# Autodesk Inventor assembly: platform
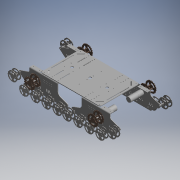
[picture p0: Inventor's stored thumbnail of the model, 180x180]
Saved by Autodesk Inventor 2019.4 (Build 234330000, 330)
## iProperties
Part Number: platform
Document SubType Name: Assembly
Designer: Jorge
Author: Jorge
## Documents named in this file (7)
- D:\TFG\dev\hardware\ROVER\platform.iam
- D:\TFG\dev\hardware\ROVER\platform_board.ipt
- D:\TFG\dev\hardware\ROVER\platform_track_support.ipt
- D:\TFG\dev\hardware\ROVER\platform_track_support_inv.ipt
- D:\TFG\dev\hardware\ROVER\platform_motor.ipt
- D:\TFG\dev\hardware\ROVER\platform_wheel.ipt
- D:\TFG\dev\hardware\ROVER\platform_sprocket.ipt
## Components (33 placed, 6 different names)
1. platform_board:1 — Mate:1, Mate:2, Mate:3, Mate:4, Mate:5, Mate:6, Mate:7, Mate:8, Mate:9, Mate:10, Mate:11, Mate:12, Mate:25, Mate:26, Mate:27
2. platform_track_support:1 — Mate:3, Mate:9, Mate:10, Mate:18, Mate:19, Mate:20, Mate:36, Mate:37, Mate:38, Mate:39, Mate:40, Mate:41, Mate:42, Mate:43, Mate:46, Mate:47
3. platform_track_support:2 — Mate:1, Mate:5, Mate:6, Mate:21, Mate:22, Mate:23, Mate:53, Mate:54, Mate:55, Mate:56, Mate:57, Mate:63, Mate:64, Mate:65, Mate:66, Mate:67
4. platform_track_support_inv:1 — Mate:4, Mate:7, Mate:8, Mate:13, Mate:14, Mate:15, Mate:48, Mate:49, Mate:50, Mate:51, Mate:52, Mate:58, Mate:59, Mate:60, Mate:61, Mate:62
5. platform_track_support_inv:2 — Mate:2, Mate:11, Mate:12, Mate:16, Mate:17, Mate:24, Mate:28, Mate:29, Mate:30, Mate:31, Mate:32, Mate:33, Mate:34, Mate:35, Mate:44, Mate:45
6. platform_motor:1 — Mate:13, Mate:14, Mate:15, Mate:71, Mate:72
7. platform_motor:2 — Mate:18, Mate:19, Mate:20, Mate:69, Mate:70
8. platform_motor:3 — Mate:16, Mate:17, Mate:24, Mate:74, Flush:1
9. platform_motor:4 — Mate:21, Mate:22, Mate:23, Mate:73
10. platform_wheel:1 — Mate:28, Mate:29
11. platform_wheel:2 — Mate:31, Mate:34
12. platform_wheel:3 — Mate:30, Mate:35
13. platform_wheel:4 — Mate:32, Mate:33
14. platform_wheel:5 — Mate:36, Mate:37
15. platform_wheel:6 — Mate:38, Mate:41
16. platform_wheel:7 — Mate:39, Mate:42
17. platform_wheel:8 — Mate:40, Mate:43
18. platform_wheel:9 — Mate:46, Mate:47
19. platform_wheel:10 — Mate:44, Mate:45
20. platform_wheel:11 — Mate:49, Mate:59
21. platform_wheel:12 — Mate:50, Mate:60
22. platform_wheel:13 — Mate:51, Mate:61
23. platform_wheel:14 — Mate:52, Mate:62
24. platform_wheel:15 — Mate:53, Mate:67
25. platform_wheel:16 — Mate:54, Mate:66
26. platform_wheel:17 — Mate:55, Mate:65
27. platform_wheel:18 — Mate:56, Mate:64
28. platform_wheel:19 — Mate:57, Mate:63
29. platform_wheel:20 — Mate:48, Mate:58
30. platform_sprocket:1 — Mate:74, Flush:1
31. platform_sprocket:2 — Mate:69, Mate:70
32. platform_sprocket:3 — Mate:71, Mate:72
33. platform_sprocket:4 — Mate:73
## Relationships (74: Mate 73, Flush 1)
- Mate:1: platform_board:1 ↔ platform_track_support:2
- Mate:2: platform_board:1 ↔ platform_track_support_inv:2
- Mate:3: platform_board:1 ↔ platform_track_support:1
- Mate:4: platform_board:1 ↔ platform_track_support_inv:1
- Mate:5: platform_board:1 ↔ platform_track_support:2
- Mate:6: platform_board:1 ↔ platform_track_support:2
- Mate:7: platform_board:1 ↔ platform_track_support_inv:1
- Mate:8: platform_board:1 ↔ platform_track_support_inv:1
- Mate:9: platform_board:1 ↔ platform_track_support:1
- Mate:10: platform_board:1 ↔ platform_track_support:1
- Mate:11: platform_board:1 ↔ platform_track_support_inv:2
- Mate:12: platform_board:1 ↔ platform_track_support_inv:2
- Mate:13: platform_track_support_inv:1 ↔ platform_motor:1
- Mate:14: platform_track_support_inv:1 ↔ platform_motor:1
- Mate:15: platform_track_support_inv:1 ↔ platform_motor:1
- Mate:16: platform_track_support_inv:2 ↔ platform_motor:3
- Mate:17: platform_track_support_inv:2 ↔ platform_motor:3
- Mate:18: platform_track_support:1 ↔ platform_motor:2
- Mate:19: platform_track_support:1 ↔ platform_motor:2
- Mate:20: platform_track_support:1 ↔ platform_motor:2
- Mate:21: platform_track_support:2 ↔ platform_motor:4
- Mate:22: platform_track_support:2 ↔ platform_motor:4
- Mate:23: platform_track_support:2 ↔ platform_motor:4
- Mate:24: platform_track_support_inv:2 ↔ platform_motor:3
- Mate:25: platform_board:1
- Mate:26: platform_board:1
- Mate:27: platform_board:1
- Mate:28: platform_track_support_inv:2 ↔ platform_wheel:1
- Mate:29: platform_track_support_inv:2 ↔ platform_wheel:1
- Mate:30: platform_track_support_inv:2 ↔ platform_wheel:3
- Mate:31: platform_track_support_inv:2 ↔ platform_wheel:2
- Mate:32: platform_track_support_inv:2 ↔ platform_wheel:4
- Mate:33: platform_track_support_inv:2 ↔ platform_wheel:4
- Mate:34: platform_track_support_inv:2 ↔ platform_wheel:2
- Mate:35: platform_track_support_inv:2 ↔ platform_wheel:3
- Mate:36: platform_track_support:1 ↔ platform_wheel:5
- Mate:37: platform_track_support:1 ↔ platform_wheel:5
- Mate:38: platform_track_support:1 ↔ platform_wheel:6
- Mate:39: platform_track_support:1 ↔ platform_wheel:7
- Mate:40: platform_track_support:1 ↔ platform_wheel:8
- Mate:41: platform_track_support:1 ↔ platform_wheel:6
- Mate:42: platform_track_support:1 ↔ platform_wheel:7
- Mate:43: platform_track_support:1 ↔ platform_wheel:8
- Mate:44: platform_track_support_inv:2 ↔ platform_wheel:10
- Mate:45: platform_track_support_inv:2 ↔ platform_wheel:10
- Mate:46: platform_track_support:1 ↔ platform_wheel:9
- Mate:47: platform_track_support:1 ↔ platform_wheel:9
- Mate:48: platform_track_support_inv:1 ↔ platform_wheel:20
- Mate:49: platform_track_support_inv:1 ↔ platform_wheel:11
- Mate:50: platform_track_support_inv:1 ↔ platform_wheel:12
- Mate:51: platform_track_support_inv:1 ↔ platform_wheel:13
- Mate:52: platform_track_support_inv:1 ↔ platform_wheel:14
- Mate:53: platform_track_support:2 ↔ platform_wheel:15
- Mate:54: platform_track_support:2 ↔ platform_wheel:16
- Mate:55: platform_track_support:2 ↔ platform_wheel:17
- Mate:56: platform_track_support:2 ↔ platform_wheel:18
- Mate:57: platform_track_support:2 ↔ platform_wheel:19
- Mate:58: platform_track_support_inv:1 ↔ platform_wheel:20
- Mate:59: platform_track_support_inv:1 ↔ platform_wheel:11
- Mate:60: platform_track_support_inv:1 ↔ platform_wheel:12
- Mate:61: platform_track_support_inv:1 ↔ platform_wheel:13
- Mate:62: platform_track_support_inv:1 ↔ platform_wheel:14
- Mate:63: platform_track_support:2 ↔ platform_wheel:19
- Mate:64: platform_track_support:2 ↔ platform_wheel:18
- Mate:65: platform_track_support:2 ↔ platform_wheel:17
- Mate:66: platform_track_support:2 ↔ platform_wheel:16
- Mate:67: platform_track_support:2 ↔ platform_wheel:15
- Mate:69: platform_motor:2 ↔ platform_sprocket:2
- Mate:70 (15 mm): platform_motor:2 ↔ platform_sprocket:2
- Mate:71: platform_motor:1 ↔ platform_sprocket:3
- Mate:72 (-15 mm): platform_motor:1 ↔ platform_sprocket:3
- Mate:73: platform_motor:4 ↔ platform_sprocket:4
- Mate:74: platform_motor:3 ↔ platform_sprocket:1
- Flush:1 (-10 mm): platform_motor:3 ↔ platform_sprocket:1
